# Autodesk Inventor assembly: GP5-300
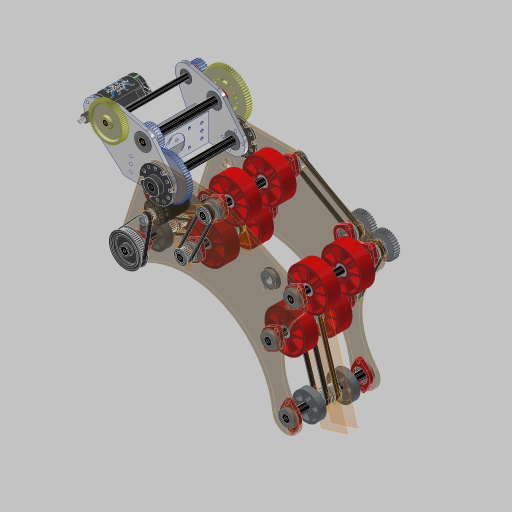
[picture p0: Inventor's stored thumbnail of the model, 512x512]
Saved by Autodesk Inventor 2023.5 (Build 275446000, 446)
## iProperties
Created: 2025-02-06
Part Number: GP5-300
Document SubType Name: Assembly
Designer: slick
Mass: 4900.96 g
Surface Area: 10054.9 cm^2
Volume: 2023.21 cm^3
Density: 2.42236 g/cm^3
Author: slick
## Documents named in this file (3)
- C:\Users\slick\OneDrive\Desktop\2025-ReefScape---CAD\Gripper\GP5\GP5-300.iam
- C:\Users\slick\OneDrive\Desktop\2025-ReefScape---CAD\Gripper\GP5\GP5-200.iam
- C:\Users\slick\OneDrive\Desktop\2025-ReefScape---CAD\Gripper\GP5\GP5-100-TAV.iam
## Components (2 placed, 2 different names)
1. GP5-200:1 [sub-assembly] — Mate:1, Mate:2, Angle:1
2. GP5-100-TAV:1 [sub-assembly] — Mate:1, Mate:2, Angle:1
## Relationships (3: Mate 2, Angle 1)
- Mate:1: GP5-200:1 ↔ GP5-100-TAV:1
- Mate:2: GP5-200:1 ↔ GP5-100-TAV:1
- Angle:1 (0 deg): GP5-200:1 ↔ GP5-100-TAV:1
